# Autodesk Inventor assembly: Clamp(maxOpening18mm)-sample
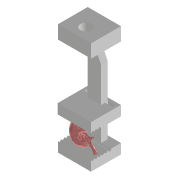
[picture p0: Inventor's stored thumbnail of the model, 180x180]
Saved by Autodesk Inventor 2021 (Build 250183000, 183)
## iProperties
Created: 2023-02-13
Part Number: Clamp(maxOpening18mm)-sample
Document SubType Name: Assembly
Designer: nvladi
Author: nvladi
## Documents named in this file (4)
- C:\Users\Public\GitHub-public\benchtop-hardware\Benchtop\CAD-model-Inventor2021\mesoSPIM\sample_handling\assemblies\Clamp(maxOpening18mm)-sample.iam
- C:\Users\Public\GitHub-public\benchtop-hardware\Benchtop\CAD-model-Inventor2021\mesoSPIM\sample_handling\cuvette-clamps\Cuvette-7.5x12.5mm(UG203)\kidney-7mm.ipt
- C:\Users\Public\GitHub-public\benchtop-hardware\Benchtop\CAD-model-Inventor2021\mesoSPIM\sample_handling\sample-holders\Clamp-part1-base9x10mm-narrowTOP.ipt
- C:\Users\Public\GitHub-public\benchtop-hardware\Benchtop\CAD-model-Inventor2021\mesoSPIM\sample_handling\sample-holders\Clamp-part2(moving)-Base9x10mm_100913(01)_C.ipt
## Components (3 placed, 3 different names)
1. kidney-7mm:1
2. Clamp-part1-base9x10mm-narrowTOP:1 — Mate:1, Mate:2
3. Clamp-part2(moving)-Base9x10mm_100913(01)_C:1 — Mate:1, Mate:2
## Relationships (2: Mate 2)
- Mate:1: Clamp-part1-base9x10mm-narrowTOP:1 ↔ Clamp-part2(moving)-Base9x10mm_100913(01)_C:1
- Mate:2: Clamp-part1-base9x10mm-narrowTOP:1 ↔ Clamp-part2(moving)-Base9x10mm_100913(01)_C:1
